# Autodesk Inventor assembly: PartsAssembly
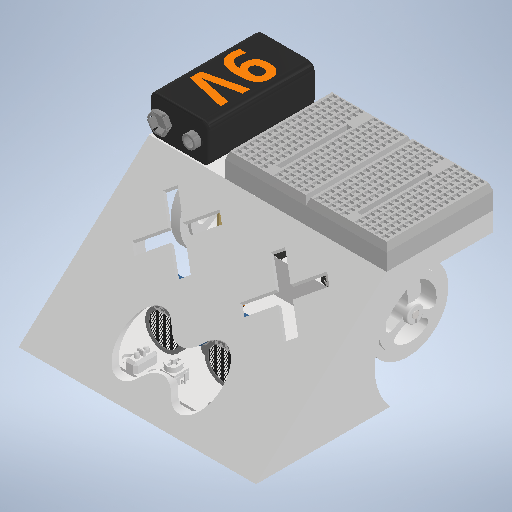
[picture p0: Inventor's stored thumbnail of the model, 512x512]
Saved by Autodesk Inventor 2025.1 (Build 291241020, 241B)
## iProperties
Created: 2024-12-27
Part Number: PartsAssembly
Document SubType Name: Assembly
Designer: herme
Author: herme
## Documents named in this file (8)
- C:\Users\herme\Documents\Sumobot\CAD\PartsAssembly.iam
- C:\Users\herme\Documents\Sumobot\CAD\Kit Parts\Motor.iam
- C:\Users\herme\Documents\Sumobot\CAD\Kit Parts\Wheel 34mm.ipt
- C:\Users\herme\Documents\Sumobot\CAD\Kit Parts\IRSensor.ipt
- C:\Users\herme\Documents\Sumobot\CAD\Kit Parts\UltrasonicSensor.iam
- C:\Users\herme\Documents\Sumobot\CAD\Shell.ipt
- C:\Users\herme\Documents\Sumobot\CAD\Kit Parts\Breadboard.ipt
- C:\Users\herme\Documents\Sumobot\CAD\Kit Parts\9VBattery.ipt
## Components (10 placed, 7 different names)
1. Wheel 34mm:1 — Insert:2
2. Wheel 34mm:2 — Insert:1
3. Motor:1 [sub-assembly] — Insert:1, Mate:1, Mate:7, Tangent:2
4. Motor:2 [sub-assembly] — Insert:2, Mate:2, Mate:8, Tangent:1
5. IRSensor:2 — Mate:12, Mate:13, Mate:14
6. UltrasonicSensor:1 [sub-assembly] — Mate:9, Mate:10, Mate:11, Flush:7
7. Shell:1 — Flush:1, Mate:1, Mate:2, Mate:4, Mate:5, Flush:4, Mate:6, Flush:5, Flush:6, Mate:7, Mate:8, Tangent:1, Tangent:2, Mate:9, Mate:10, Mate:11, Flush:7, Mate:12, Mate:13, Mate:14
8. Breadboard:1 — Mate:3, Flush:2, Flush:3, Mate:4, Mate:5
9. Breadboard:2 — Mate:3, Flush:2, Flush:3, Flush:4
10. 9VBattery:1 — Mate:6, Flush:5, Flush:6
## Relationships (25: Mate 14, Flush 7, Insert 2, Tangent 2)
- Insert:1: Wheel 34mm:2 ↔ Motor:1
- Insert:2: Wheel 34mm:1 ↔ Motor:2
- Flush:1: Shell:1
- Mate:1: Motor:1 ↔ Shell:1
- Mate:2: Motor:2 ↔ Shell:1
- Mate:3: Breadboard:1 ↔ Breadboard:2
- Flush:2: Breadboard:1 ↔ Breadboard:2
- Flush:3: Breadboard:1 ↔ Breadboard:2
- Mate:4: Shell:1 ↔ Breadboard:1
- Mate:5: Shell:1 ↔ Breadboard:1
- Flush:4: Shell:1 ↔ Breadboard:2
- Mate:6: Shell:1 ↔ 9VBattery:1
- Flush:5: Shell:1 ↔ 9VBattery:1
- Flush:6: Shell:1 ↔ 9VBattery:1
- Mate:7: Motor:1 ↔ Shell:1
- Mate:8: Motor:2 ↔ Shell:1
- Tangent:1 (17.5 mm): Motor:2 ↔ Shell:1
- Tangent:2 (17.5 mm): Motor:1 ↔ Shell:1
- Mate:9 (24.5 mm): UltrasonicSensor:1 ↔ Shell:1
- Mate:10: UltrasonicSensor:1 ↔ Shell:1
- Mate:11 (32.8 mm): UltrasonicSensor:1 ↔ Shell:1
- Flush:7: UltrasonicSensor:1 ↔ Shell:1
- Mate:12: IRSensor:2 ↔ Shell:1
- Mate:13 (25 mm): IRSensor:2 ↔ Shell:1
- Mate:14: IRSensor:2 ↔ Shell:1
